# Autodesk Inventor assembly: am-2598_107 2016 KOP Toughbox Mini
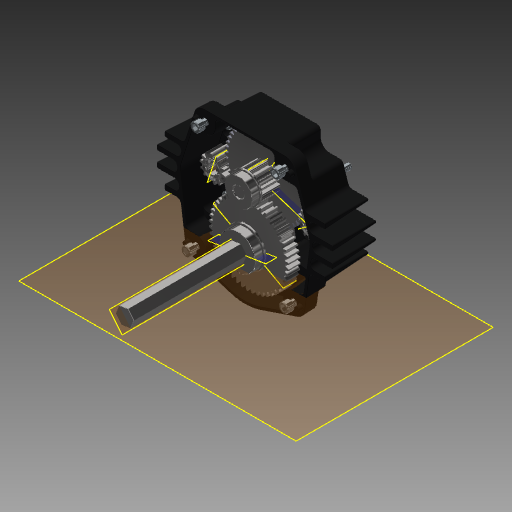
[picture p0: Inventor's stored thumbnail of the model, 512x512]
Saved by Autodesk Inventor 2017.1 (Build 211199000, 199)
## iProperties
Created: 2015-12-05
Part Number: am-2598_107 2016 KOP Toughbox Mini
Document SubType Name: Assembly
Designer: PhillipD
Author: PhillipD
Revision Number: ANY
## Documents named in this file (16)
- D:\FIRST\FIRST KOP 2017\FIRST Drive Base\Parts\am-2598_107 2016 KOP Toughbox Mini.iam
- D:\FIRST\FIRST KOP 2017\FIRST Drive Base\Parts\Toughbox d07.ipt
- D:\FIRST\FIRST KOP 2017\FIRST Drive Base\Parts\Toughbox d05.ipt
- D:\FIRST\FIRST KOP 2017\FIRST Drive Base\Parts\FR6ZZ Bearing.ipt
- D:\FIRST\FIRST KOP 2017\FIRST Drive Base\Parts\10-32 Nylock Nut.ipt
- D:\FIRST\FIRST KOP 2017\FIRST Drive Base\Parts\5-16 washer.ipt
- D:\FIRST\FIRST KOP 2017\FIRST Drive Base\Parts\Toughbox d09.ipt
- D:\FIRST\FIRST KOP 2017\FIRST Drive Base\Parts\TM Housing.ipt
- D:\FIRST\FIRST KOP 2017\FIRST Drive Base\Parts\SHCS 10-32 x 0.625.ipt
- D:\FIRST\FIRST KOP 2017\FIRST Drive Base\Parts\R6ZZ Bearing.ipt
- D:\FIRST\FIRST KOP 2017\FIRST Drive Base\Parts\8mm spring clip.ipt
- D:\FIRST\FIRST KOP 2017\FIRST Drive Base\Parts\500 E-klip.ipt
- D:\FIRST\FIRST KOP 2017\FIRST Drive Base\Parts\FR8ZZ Hex Bearing.ipt
- D:\FIRST\FIRST KOP 2017\FIRST Drive Base\Parts\16t 20dp 375h with teeth.ipt
- D:\FIRST\FIRST KOP 2017\FIRST Drive Base\Parts\48t 20dp 500h with teeth.ipt
- D:\FIRST\FIRST KOP 2017\FIRST Drive Base\Parts\TB Output Shaft Hex L-Base 2.ipt
## Components (31 placed, 31 different names)
1. Toughbox d07_15 — Mate:3, Insert:5, Angle:3
2. Toughbox d05_16 — Mate:7, Mate:8, Angle:3, Mate:14, Aligns Gear 1, Aligns Gear 2, Rotation:1
3. FR6ZZ Bearing_17 — Mate:1, Mate:2, Insert:5
4. 10-32 Nylock Nut_18
5. 10-32 Nylock Nut_19
6. 10-32 Nylock Nut_20
7. 10-32 Nylock Nut_21
8. 5-16 washer_22
9. 5-16 washer_23 — Insert:3
10. 5-16 washer_24 — Insert:4
11. 5-16 washer_25
12. Toughbox d09_26 — Insert:3, Mate:9, Mate:13, Angle:4, Aligns Gear 1, Rotation:1, Rotation:2
13. Toughbox d09_27 — Insert:4, Aligns Gear 2, Rotation:2
14. TM Housing_28
15. SHCS 10-32 x 0.625_29
16. SHCS 10-32 x 0.625_30
17. SHCS 10-32 x 0.625_31
18. SHCS 10-32 x 0.625_32
19. SHCS 10-32 x 0.625_33
20. SHCS 10-32 x 0.625_34
21. SHCS 10-32 x 0.625_35
22. SHCS 10-32 x 0.625_36
23. R6ZZ Bearing_37 — Mate:7, Mate:8, Mate:10
24. R6ZZ Bearing_38 — Insert:1
25. 8mm spring clip_39
26. 8mm spring clip_40
27. 500 E-klip_41 — Insert:2
28. FR8ZZ Hex Bearing_42 — Flush:1, Mate:4, Angle:1, Mate:6
29. 16t 20dp 375h with teeth_43 — Mate:1, Mate:2, Mate:3, Mate:15, Rotation:3
30. 48t 20dp 500h with teeth_44 — Mate:5, Angle:2, Mate:6, Mate:15, Rotation:3
31. TB Output Shaft Hex L-Base 2_45 — Insert:1, Insert:2, Flush:1, Mate:4, Angle:1, Mate:5, Angle:2
## Relationships (30: Mate 15, Angle 6, Insert 5, RelateRotation 3, Flush 1)
- Insert:1: R6ZZ Bearing_38 ↔ TB Output Shaft Hex L-Base 2_45
- Insert:2: 500 E-klip_41 ↔ TB Output Shaft Hex L-Base 2_45
- Insert:3: 5-16 washer_23 ↔ Toughbox d09_26
- Insert:4: 5-16 washer_24 ↔ Toughbox d09_27
- Mate:1: FR6ZZ Bearing_17 ↔ 16t 20dp 375h with teeth_43
- Mate:2: FR6ZZ Bearing_17 ↔ 16t 20dp 375h with teeth_43
- Mate:3: Toughbox d07_15 ↔ 16t 20dp 375h with teeth_43
- Insert:5 (0.6096 mm): Toughbox d07_15 ↔ FR6ZZ Bearing_17
- Flush:1 (-89.4334 mm): FR8ZZ Hex Bearing_42 ↔ TB Output Shaft Hex L-Base 2_45
- Mate:4: FR8ZZ Hex Bearing_42 ↔ TB Output Shaft Hex L-Base 2_45
- Angle:1 (0 deg): FR8ZZ Hex Bearing_42 ↔ TB Output Shaft Hex L-Base 2_45
- Mate:5: 48t 20dp 500h with teeth_44 ↔ TB Output Shaft Hex L-Base 2_45
- Angle:2 (0 deg): 48t 20dp 500h with teeth_44 ↔ TB Output Shaft Hex L-Base 2_45
- Mate:6 (1.1176 mm): FR8ZZ Hex Bearing_42 ↔ 48t 20dp 500h with teeth_44
- Mate:7: Toughbox d05_16 ↔ R6ZZ Bearing_37
- Mate:8: Toughbox d05_16 ↔ R6ZZ Bearing_37
- Angle:3 (0 deg): Toughbox d07_15 ↔ Toughbox d05_16
- Mate:9: Toughbox d09_26
- Mate:10: R6ZZ Bearing_37
- Mate:11
- Mate:12
- Mate:13: Toughbox d09_26
- Mate:14: Toughbox d05_16
- Angle:4 (0 deg): Toughbox d09_26
- Aligns Gear 1 [Angle] (0 deg): Toughbox d05_16 ↔ Toughbox d09_26
- Aligns Gear 2 [Angle] (35.5 deg): Toughbox d05_16 ↔ Toughbox d09_27
- Rotation:1 [RelateRotation] (0.28 ul): Toughbox d05_16 ↔ Toughbox d09_26
- Rotation:2 [RelateRotation] (1 ul): Toughbox d09_26 ↔ Toughbox d09_27
- Mate:15: 16t 20dp 375h with teeth_43 ↔ 48t 20dp 500h with teeth_44
- Rotation:3 [RelateRotation] (0.3333 ul): 16t 20dp 375h with teeth_43 ↔ 48t 20dp 500h with teeth_44
